# Autodesk Inventor assembly: intake
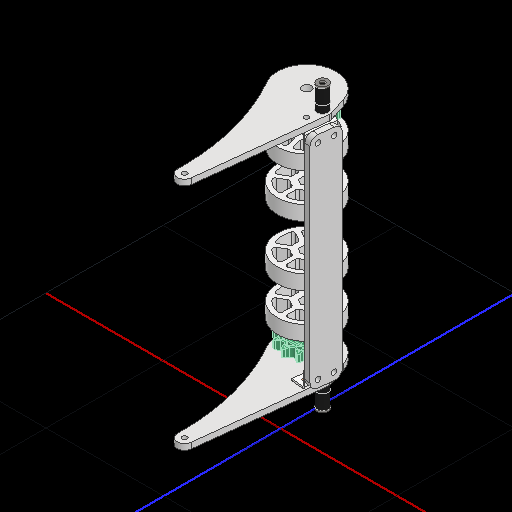
[picture p0: Inventor's stored thumbnail of the model, 512x512]
Saved by Autodesk Inventor 2025.2 (Build 292293000, 293)
## iProperties
Created: 2025-12-05
Part Number: intake
Document SubType Name: Assembly
Designer: cloudy
Author: cloudy
## Documents named in this file (13)
- C:\Users\cloudy\Documents\AURA_CAD\15\intake.iam
- C:\Users\cloudy\Documents\AURA_CAD\!lib\Motion\Wheels\Flex Wheels\2.000 Flex Wheel\2.000 30A .500.ipt
- C:\Users\cloudy\Documents\GitHub\aura-cad\!lib\Motion\Wheels\Flex Wheels\2.000 Flex Wheel.ipt
- C:\Users\cloudy\Documents\AURA_CAD\!lib\Motion\Sprockets\9P Sprocket\9P 12T Sprocket, No Insert.iam
- C:\Users\cloudy\Documents\GitHub\aura-cad\!lib\Motion\Sprockets\9P Sprocket.iam
- C:\Users\cloudy\Documents\AURA_CAD\15\intakeSide.ipt
- C:\Users\cloudy\Documents\AURA_CAD\!lib\Structure\C Channel\Aluminum 1x3x1 Half\Alu C Half 1x3x1x2.ipt
- C:\Users\cloudy\Documents\AURA_CAD\15\intakebrace.ipt
- C:\Users\cloudy\Documents\AURA_CAD\!lib\Motion\Spacers\Spacer Nylon .375 OD\NSpacer .375 OD x .500.ipt
- C:\Users\cloudy\Documents\GitHub\aura-cad\!lib\Motion\Spacers\Spacer Nylon .375 OD.ipt
- C:\Users\cloudy\Documents\AURA_CAD\!lib\Motion\Spacers\Spacer Nylon .375 OD\NSpacer .375 OD x .250.ipt
- C:\Users\cloudy\Documents\AURA_CAD\!lib\Motion\Spacers\Washer Steel\SWasher .375 OD x .062500.ipt
- C:\Users\cloudy\Documents\GitHub\aura-cad\!lib\Motion\Spacers\Washer Steel.ipt
## Components (17 placed, 8 different names)
1. 2.000 30A .500:3 — Insert:5, Insert:16
2. 2.000 30A .500:4 — Insert:5
3. intakeSide:1 — Insert:15, Insert:19, Mate:1, Insert:23
4. intakeSide:2 — Insert:20, Mate:2, Mate:3, Insert:26
5. Alu C Half 1x3x1x2:1 — Insert:20, Mate:2, Flush:1
6. 9P 12T Sprocket, No Insert:1 [sub-assembly] — Insert:14, Insert:15, Insert:16
7. 9P 12T Sprocket, No Insert:2 [sub-assembly] — Insert:14, Insert:17
8. 2.000 30A .500:5 — Insert:18
9. 2.000 30A .500:6 — Insert:17, Insert:18, Mate:3
10. Alu C Half 1x3x1x2:2 — Insert:19, Mate:1
11. intakebrace:1 — Flush:1
12. NSpacer .375 OD x .500:1 — Insert:21, Insert:22
13. NSpacer .375 OD x .250:2 — Insert:22, Insert:23
14. SWasher .375 OD x .062500:1 — Insert:21
15. NSpacer .375 OD x .500:3
16. NSpacer .375 OD x .250:4 — Insert:26
17. SWasher .375 OD x .062500:2
## Relationships (18: Insert 14, Mate 3, Flush 1)
- Insert:5 (25.4 mm): 2.000 30A .500:3 ↔ 2.000 30A .500:4
- Insert:14 (-186.69 mm): 9P 12T Sprocket, No Insert:1 ↔ 9P 12T Sprocket, No Insert:2
- Insert:15 (3.4925 mm): intakeSide:1 ↔ 9P 12T Sprocket, No Insert:1
- Insert:16 (9.525 mm): 2.000 30A .500:3 ↔ 9P 12T Sprocket, No Insert:1
- Insert:17 (9.525 mm): 9P 12T Sprocket, No Insert:2 ↔ 2.000 30A .500:6
- Insert:18 (25.4 mm): 2.000 30A .500:5 ↔ 2.000 30A .500:6
- Insert:19: intakeSide:1 ↔ Alu C Half 1x3x1x2:2
- Mate:1: intakeSide:1 ↔ Alu C Half 1x3x1x2:2
- Insert:20: intakeSide:2 ↔ Alu C Half 1x3x1x2:1
- Mate:2: intakeSide:2 ↔ Alu C Half 1x3x1x2:1
- Mate:3: intakeSide:2 ↔ 2.000 30A .500:6
- Flush:1: Alu C Half 1x3x1x2:1 ↔ intakebrace:1
- Insert:21: NSpacer .375 OD x .500:1 ↔ SWasher .375 OD x .062500:1
- Insert:22: NSpacer .375 OD x .500:1 ↔ NSpacer .375 OD x .250:2
- Insert:23: intakeSide:1 ↔ NSpacer .375 OD x .250:2
- [Insert]: NSpacer .375 OD x .500:3 ↔ SWasher .375 OD x .062500:2
- [Insert]: NSpacer .375 OD x .500:3 ↔ NSpacer .375 OD x .250:4
- Insert:26: intakeSide:2 ↔ NSpacer .375 OD x .250:4
## Named parameters: d65_d62 = 0 mm, d66_d63 = 0 mm
